# Autodesk Inventor assembly: Steam Engine 2 inch
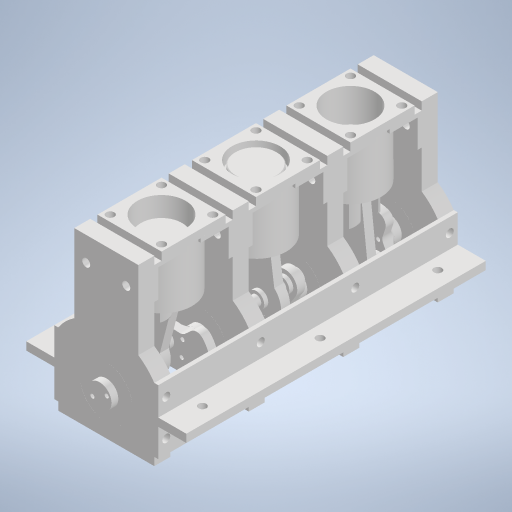
[picture p0: Inventor's stored thumbnail of the model, 512x512]
Saved by Autodesk Inventor 2023 (Build 270158000, 158)
## iProperties
Created: 2022-10-29
Part Number: Steam Engine 2 inch
Document SubType Name: Assembly
Designer: tommy
Author: tommy
## Documents named in this file (16)
- C:\Users\tommy\Documents\Repositories\Steam Engine\2 inch Design\Steam Engine 2 inch.iam
- C:\Users\tommy\Documents\Repositories\Steam Engine\2 inch Design\Wrist Pin Bearing.ipt
- C:\Users\tommy\Documents\Repositories\Steam Engine\2 inch Design\Wrist Pin.ipt
- C:\Users\tommy\Documents\Repositories\Steam Engine\2 inch Design\Piston O Ring.ipt
- C:\Users\tommy\Documents\Repositories\Steam Engine\2 inch Design\Connecting Rod.ipt
- C:\Users\tommy\Documents\Repositories\Steam Engine\2 inch Design\Cylinder Bracket.ipt
- C:\Users\tommy\Documents\Repositories\Steam Engine\2 inch Design\Connecting Rod Bearing.ipt
- C:\Users\tommy\Documents\Repositories\Steam Engine\2 inch Design\Cylinders.ipt
- C:\Users\tommy\Documents\Repositories\Steam Engine\2 inch Design\Piston Head.ipt
- C:\Users\tommy\Documents\Repositories\Steam Engine\2 inch Design\CrankShaft Main Bearing.ipt
- C:\Users\tommy\Documents\Repositories\Steam Engine\2 inch Design\Frame Middle.ipt
- C:\Users\tommy\Documents\Repositories\Steam Engine\2 inch Design\Frame Bottom.ipt
- C:\Users\tommy\Documents\Repositories\Steam Engine\2 inch Design\Crank on Crankshaft.ipt
- C:\Users\tommy\Documents\Repositories\Steam Engine\2 inch Design\Crankshaft.ipt
- C:\Users\tommy\Documents\Repositories\Steam Engine\2 inch Design\Crankshaft Crank Cylinder.ipt
- C:\Users\tommy\Documents\Repositories\Steam Engine\2 inch Design\Frame Bracket.ipt
## Components (59 placed, 15 different names)
1. Connecting Rod:2
2. Piston O Ring:3
3. Piston O Ring:4
4. Cylinder Bracket:3
5. Cylinder Bracket:4 — Mate:120, Mate:121, Mate:122
6. Connecting Rod Bearing:2
7. Wrist Pin Bearing:2
8. Wrist Pin:2
9. Cylinders:2
10. Piston Head:2
11. CrankShaft Main Bearing:3
12. Frame Middle:2 — Mate:84, Mate:85, Mate:86, Mate:138
13. Frame Bottom:2
14. Crank on Crankshaft:3 — Mate:123, Mate:124
15. Crank on Crankshaft:4
16. Crankshaft Crank Cylinder:2
17. Crankshaft:3 — Mate:125, Mate:126
18. Connecting Rod:3
19. Piston O Ring:5
20. Piston O Ring:6
21. Cylinder Bracket:5
22. Cylinder Bracket:6 — Mate:130, Mate:131, Mate:132
23. Connecting Rod Bearing:3
24. Wrist Pin Bearing:3
25. Wrist Pin:3
26. Cylinders:3
27. Piston Head:3
28. CrankShaft Main Bearing:4
29. Frame Middle:3 — Mate:120, Mate:121, Mate:122, Mate:139
30. Frame Bottom:3
31. Crank on Crankshaft:5 — Mate:147, Mate:148, Mate:149
32. Crank on Crankshaft:6
33. Crankshaft Crank Cylinder:3
34. Crankshaft:4 — Mate:123, Mate:124
35. CrankShaft Main Bearing:5 — Mate:150
36. Frame Middle:4 — Mate:130, Mate:131, Mate:132, Mate:140, Mate:144, Mate:146
37. Frame Bottom:4
38. Frame Bracket:1 — Mate:133, Mate:134, Mate:135
39. Frame Bracket:2 — Mate:133, Mate:134, Mate:135, Mate:136, Mate:137, Mate:138, Mate:139, Mate:140
40. Frame Bracket:3 — Mate:144
41. Frame Bracket:4 — Mate:145, Mate:146
42. Crankshaft:5 — Mate:147, Mate:148, Mate:149, Mate:150
43. Connecting Rod:1 — Flush:1, Mate:8, Mate:10, Flush:2, Mate:36
44. Piston O Ring:1 — Tangent:2, Mate:11
45. Piston O Ring:2 — Tangent:1, Mate:12
46. Cylinder Bracket:1 — Mate:1, Mate:2, Mate:3, Mate:38, Mate:39, Mate:40
47. Cylinder Bracket:2 — Mate:4, Mate:5, Mate:6, Mate:84, Mate:85, Mate:86
48. Connecting Rod Bearing:1 — Mate:10, Flush:2, Mate:37
49. Wrist Pin Bearing:1 — Mate:7, Flush:1, Mate:8, Mate:9
50. Wrist Pin:1 — Mate:7, Mate:9, Mate:13, Mate:14
51. Cylinders:1 — Mate:1, Mate:2, Mate:3, Mate:4, Mate:5, Mate:6, Mate:21
52. Piston Head:1 — Tangent:1, Tangent:2, Mate:11, Mate:12, Mate:13, Mate:14, Mate:21
53. CrankShaft Main Bearing:2 — Mate:41, Mate:42, Mate:50
54. Frame Middle:1 — Mate:38, Mate:39, Mate:40, Mate:41, Mate:42, Mate:43, Flush:3, Flush:4, Mate:136, Mate:137, Mate:145
55. Frame Bottom:1 — Mate:43, Flush:3, Flush:4
56. Crank on Crankshaft:1 — Mate:32, Mate:34, Mate:125, Mate:126
57. Crank on Crankshaft:2 — Mate:33, Mate:35, Mate:47, Mate:48, Mate:49
58. Crankshaft Crank Cylinder:1 — Mate:32, Mate:33, Mate:34, Mate:35, Mate:36, Mate:37
59. Crankshaft:2 — Mate:47, Mate:48, Mate:49, Mate:50
## Relationships (147: Mate 127, Flush 14, Tangent 6)
- Mate:1: Cylinder Bracket:1 ↔ Cylinders:1
- Mate:2: Cylinder Bracket:1 ↔ Cylinders:1
- Mate:3: Cylinder Bracket:1 ↔ Cylinders:1
- Mate:4: Cylinder Bracket:2 ↔ Cylinders:1
- Mate:5: Cylinder Bracket:2 ↔ Cylinders:1
- Mate:6: Cylinder Bracket:2 ↔ Cylinders:1
- Mate:7: Wrist Pin Bearing:1 ↔ Wrist Pin:1
- Flush:1: Connecting Rod:1 ↔ Wrist Pin Bearing:1
- Mate:8: Connecting Rod:1 ↔ Wrist Pin Bearing:1
- Mate:9: Wrist Pin Bearing:1 ↔ Wrist Pin:1
- Mate:10: Connecting Rod:1 ↔ Connecting Rod Bearing:1
- Flush:2 (0.127 mm): Connecting Rod:1 ↔ Connecting Rod Bearing:1
- Tangent:1: Piston O Ring:2 ↔ Piston Head:1
- Tangent:2: Piston O Ring:1 ↔ Piston Head:1
- Mate:11: Piston O Ring:1 ↔ Piston Head:1
- Mate:12: Piston O Ring:2 ↔ Piston Head:1
- Mate:13: Wrist Pin:1 ↔ Piston Head:1
- Mate:14: Wrist Pin:1 ↔ Piston Head:1
- Mate:21: Cylinders:1 ↔ Piston Head:1
- Mate:32: Crank on Crankshaft:1 ↔ Crankshaft Crank Cylinder:1
- Mate:33: Crank on Crankshaft:2 ↔ Crankshaft Crank Cylinder:1
- Mate:34: Crank on Crankshaft:1 ↔ Crankshaft Crank Cylinder:1
- Mate:35: Crank on Crankshaft:2 ↔ Crankshaft Crank Cylinder:1
- Mate:36: Connecting Rod:1 ↔ Crankshaft Crank Cylinder:1
- Mate:37: Connecting Rod Bearing:1 ↔ Crankshaft Crank Cylinder:1
- Mate:38: Cylinder Bracket:1 ↔ Frame Middle:1
- Mate:39: Cylinder Bracket:1 ↔ Frame Middle:1
- Mate:40: Cylinder Bracket:1 ↔ Frame Middle:1
- Mate:41: CrankShaft Main Bearing:2 ↔ Frame Middle:1
- Mate:42: CrankShaft Main Bearing:2 ↔ Frame Middle:1
- Mate:43: Frame Middle:1 ↔ Frame Bottom:1
- Flush:3: Frame Middle:1 ↔ Frame Bottom:1
- Flush:4: Frame Middle:1 ↔ Frame Bottom:1
- Mate:47: Crank on Crankshaft:2 ↔ Crankshaft:2
- Mate:48: Crank on Crankshaft:2 ↔ Crankshaft:2
- Mate:49: Crank on Crankshaft:2 ↔ Crankshaft:2
- Mate:50: CrankShaft Main Bearing:2 ↔ Crankshaft:2
- [Mate]: Cylinder Bracket:3 ↔ Cylinders:2
- [Mate]: Cylinder Bracket:3 ↔ Cylinders:2
- [Mate]: Cylinder Bracket:3 ↔ Cylinders:2
- [Mate]: Cylinder Bracket:4 ↔ Cylinders:2
- [Mate]: Cylinder Bracket:4 ↔ Cylinders:2
- [Mate]: Cylinder Bracket:4 ↔ Cylinders:2
- [Mate]: Wrist Pin Bearing:2 ↔ Wrist Pin:2
- [Flush]: Connecting Rod:2 ↔ Wrist Pin Bearing:2
- [Mate]: Connecting Rod:2 ↔ Wrist Pin Bearing:2
- [Mate]: Wrist Pin Bearing:2 ↔ Wrist Pin:2
- [Mate]: Connecting Rod:2 ↔ Connecting Rod Bearing:2
- [Flush] (0.127 mm): Connecting Rod:2 ↔ Connecting Rod Bearing:2
- [Tangent]: Piston O Ring:4 ↔ Piston Head:2
- [Tangent]: Piston O Ring:3 ↔ Piston Head:2
- [Mate]: Piston O Ring:3 ↔ Piston Head:2
- [Mate]: Piston O Ring:4 ↔ Piston Head:2
- [Mate]: Wrist Pin:2 ↔ Piston Head:2
- [Mate]: Wrist Pin:2 ↔ Piston Head:2
- [Mate]: Cylinders:2 ↔ Piston Head:2
- [Mate]: Crank on Crankshaft:3 ↔ Crankshaft Crank Cylinder:2
- [Mate]: Crank on Crankshaft:4 ↔ Crankshaft Crank Cylinder:2
- [Mate]: Crank on Crankshaft:3 ↔ Crankshaft Crank Cylinder:2
- [Mate]: Crank on Crankshaft:4 ↔ Crankshaft Crank Cylinder:2
- [Mate]: Connecting Rod:2 ↔ Crankshaft Crank Cylinder:2
- [Mate]: Connecting Rod Bearing:2 ↔ Crankshaft Crank Cylinder:2
- [Mate]: Cylinder Bracket:3 ↔ Frame Middle:2
- [Mate]: Cylinder Bracket:3 ↔ Frame Middle:2
- [Mate]: Cylinder Bracket:3 ↔ Frame Middle:2
- [Mate]: CrankShaft Main Bearing:3 ↔ Frame Middle:2
- [Mate]: CrankShaft Main Bearing:3 ↔ Frame Middle:2
- [Mate]: Frame Middle:2 ↔ Frame Bottom:2
- [Flush]: Frame Middle:2 ↔ Frame Bottom:2
- [Flush]: Frame Middle:2 ↔ Frame Bottom:2
- [Mate]: Crank on Crankshaft:4 ↔ Crankshaft:3
- [Mate]: Crank on Crankshaft:4 ↔ Crankshaft:3
- [Mate]: Crank on Crankshaft:4 ↔ Crankshaft:3
- [Mate]: CrankShaft Main Bearing:3 ↔ Crankshaft:3
- Mate:84: Frame Middle:2 ↔ Cylinder Bracket:2
- Mate:85: Frame Middle:2 ↔ Cylinder Bracket:2
- Mate:86: Frame Middle:2 ↔ Cylinder Bracket:2
- [Mate]: Cylinder Bracket:5 ↔ Cylinders:3
- [Mate]: Cylinder Bracket:5 ↔ Cylinders:3
- [Mate]: Cylinder Bracket:5 ↔ Cylinders:3
- [Mate]: Cylinder Bracket:6 ↔ Cylinders:3
- [Mate]: Cylinder Bracket:6 ↔ Cylinders:3
- [Mate]: Cylinder Bracket:6 ↔ Cylinders:3
- [Mate]: Wrist Pin Bearing:3 ↔ Wrist Pin:3
- [Flush]: Connecting Rod:3 ↔ Wrist Pin Bearing:3
- [Mate]: Connecting Rod:3 ↔ Wrist Pin Bearing:3
- [Mate]: Wrist Pin Bearing:3 ↔ Wrist Pin:3
- [Mate]: Connecting Rod:3 ↔ Connecting Rod Bearing:3
- [Flush] (0.127 mm): Connecting Rod:3 ↔ Connecting Rod Bearing:3
- [Tangent]: Piston O Ring:6 ↔ Piston Head:3
- [Tangent]: Piston O Ring:5 ↔ Piston Head:3
- [Mate]: Piston O Ring:5 ↔ Piston Head:3
- [Mate]: Piston O Ring:6 ↔ Piston Head:3
- [Mate]: Wrist Pin:3 ↔ Piston Head:3
- [Mate]: Wrist Pin:3 ↔ Piston Head:3
- [Mate]: Cylinders:3 ↔ Piston Head:3
- [Mate]: Crank on Crankshaft:5 ↔ Crankshaft Crank Cylinder:3
- [Mate]: Crank on Crankshaft:6 ↔ Crankshaft Crank Cylinder:3
- [Mate]: Crank on Crankshaft:5 ↔ Crankshaft Crank Cylinder:3
- [Mate]: Crank on Crankshaft:6 ↔ Crankshaft Crank Cylinder:3
- [Mate]: Connecting Rod:3 ↔ Crankshaft Crank Cylinder:3
- [Mate]: Connecting Rod Bearing:3 ↔ Crankshaft Crank Cylinder:3
- [Mate]: Cylinder Bracket:5 ↔ Frame Middle:3
- [Mate]: Cylinder Bracket:5 ↔ Frame Middle:3
- [Mate]: Cylinder Bracket:5 ↔ Frame Middle:3
- [Mate]: CrankShaft Main Bearing:4 ↔ Frame Middle:3
- [Mate]: CrankShaft Main Bearing:4 ↔ Frame Middle:3
- [Mate]: Frame Middle:3 ↔ Frame Bottom:3
- [Flush]: Frame Middle:3 ↔ Frame Bottom:3
- [Flush]: Frame Middle:3 ↔ Frame Bottom:3
- [Mate]: Crank on Crankshaft:6 ↔ Crankshaft:4
- [Mate]: Crank on Crankshaft:6 ↔ Crankshaft:4
- [Mate]: Crank on Crankshaft:6 ↔ Crankshaft:4
- [Mate]: CrankShaft Main Bearing:4 ↔ Crankshaft:4
- Mate:120: Cylinder Bracket:4 ↔ Frame Middle:3
- Mate:121: Cylinder Bracket:4 ↔ Frame Middle:3
- Mate:122: Cylinder Bracket:4 ↔ Frame Middle:3
- Mate:123: Crank on Crankshaft:3 ↔ Crankshaft:4
- Mate:124: Crank on Crankshaft:3 ↔ Crankshaft:4
- Mate:125: Crankshaft:3 ↔ Crank on Crankshaft:1
- Mate:126: Crankshaft:3 ↔ Crank on Crankshaft:1
- [Mate]: CrankShaft Main Bearing:5 ↔ Frame Middle:4
- [Mate]: CrankShaft Main Bearing:5 ↔ Frame Middle:4
- [Mate]: Frame Middle:4 ↔ Frame Bottom:4
- [Flush]: Frame Middle:4 ↔ Frame Bottom:4
- [Flush]: Frame Middle:4 ↔ Frame Bottom:4
- Mate:130: Cylinder Bracket:6 ↔ Frame Middle:4
- Mate:131: Cylinder Bracket:6 ↔ Frame Middle:4
- Mate:132: Cylinder Bracket:6 ↔ Frame Middle:4
- Mate:133: Frame Bracket:1 ↔ Frame Bracket:2
- Mate:134: Frame Bracket:1 ↔ Frame Bracket:2
- Mate:135: Frame Bracket:1 ↔ Frame Bracket:2
- Mate:136: Frame Bracket:2 ↔ Frame Middle:1
- Mate:137: Frame Bracket:2 ↔ Frame Middle:1
- Mate:138: Frame Middle:2 ↔ Frame Bracket:2
- Mate:139: Frame Middle:3 ↔ Frame Bracket:2
- Mate:140: Frame Middle:4 ↔ Frame Bracket:2
- [Mate]: Frame Bracket:3 ↔ Frame Bracket:4
- [Mate]: Frame Bracket:3 ↔ Frame Bracket:4
- [Mate]: Frame Bracket:3 ↔ Frame Bracket:4
- Mate:144: Frame Middle:4 ↔ Frame Bracket:3
- Mate:145: Frame Bracket:4 ↔ Frame Middle:1
- Mate:146: Frame Middle:4 ↔ Frame Bracket:4
- Mate:147: Crank on Crankshaft:5 ↔ Crankshaft:5
- Mate:148: Crank on Crankshaft:5 ↔ Crankshaft:5
- Mate:149: Crank on Crankshaft:5 ↔ Crankshaft:5
- Mate:150: CrankShaft Main Bearing:5 ↔ Crankshaft:5
## Named parameters: d175_d9 = 0 mm, d176_d10 = 0 mm, d177_d11 = 0 mm, d178_d12 = 0 mm, d179_d13 = 0 mm, d180_d73 = 0 mm, d181_d74 = 0 mm, d182_d84 = 0 mm, d183_d85 = 0 mm, d184_d86 = 0 mm, d185_d87 = 0 mm, d186_d14 = 0 mm, d187_d15 = 0 mm, d188_d17 = 0 mm, d189_d18 = 0 mm, d190_d19 = 0 mm, d191_d20 = 0 mm, d192_d21 = 0.127 mm, d193_d22 = 0 mm, d194_d23 = 0 mm, d195_d24 = 0 mm, d196_d25 = 0 mm, d197_d26 = 0 mm, d198_d27 = 0 mm, d199_d42 = 0 mm, d200_d59 = 0 mm, d201_d61 = 0 mm, d202_d62 = 0 mm, d203_d63 = 0 mm, d204_d64 = 0 mm, d205_d65 = 0 mm, d206_d67 = 0 mm, d207_d68 = 0 mm, d208_d69 = 0 mm, d209_d70 = 0 mm, d210_d71 = 0 mm, d211_d72 = 0 mm, d217_d9 = 0 mm, d218_d10 = 0 mm, d219_d11 = 0 mm, d220_d12 = 0 mm, d221_d13 = 0 mm, d222_d73 = 0 mm, d223_d74 = 0 mm, d224_d84 = 0 mm, d225_d85 = 0 mm, d226_d86 = 0 mm, d227_d87 = 0 mm, d228_d14 = 0 mm, d229_d15 = 0 mm, d230_d17 = 0 mm, d231_d18 = 0 mm, d232_d19 = 0 mm, d233_d20 = 0 mm, d234_d21 = 0.127 mm, d235_d22 = 0 mm, d236_d23 = 0 mm, d237_d24 = 0 mm, d238_d25 = 0 mm, d239_d26 = 0 mm, d240_d27 = 0 mm, d241_d42 = 0 mm, d242_d59 = 0 mm, d243_d61 = 0 mm, d244_d62 = 0 mm, d245_d63 = 0 mm, d246_d64 = 0 mm, d247_d65 = 0 mm, d248_d67 = 0 mm, d249_d68 = 0 mm, d250_d69 = 0 mm, d251_d70 = 0 mm, d252_d71 = 0 mm, d253_d72 = 0 mm, d263_d73 = 0 mm, d264_d74 = 0 mm, d265_d70 = 0 mm, d266_d71 = 0 mm, d267_d72 = 0 mm, d280_d271 = 0 mm, d281_d272 = 0 mm, d282_d273 = 0 mm
